# Autodesk Inventor assembly: CARCASA_ESTRUCTURA_Y_CHAPAS
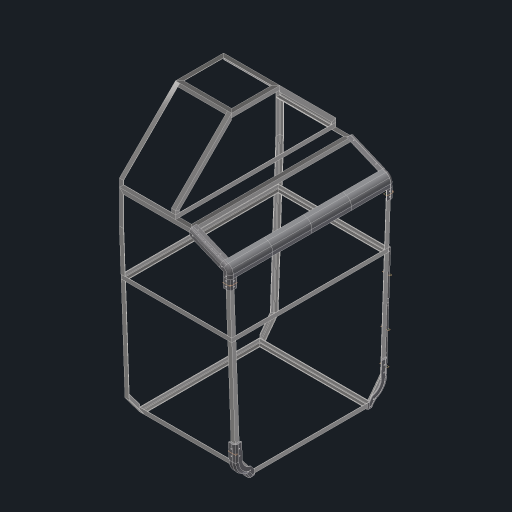
[picture p0: Inventor's stored thumbnail of the model, 512x512]
Saved by Autodesk Inventor 2024.3 (Build 283343000, 343)
## iProperties
Created: 2024-05-18
Part Number: CARCASA_ESTRUCTURA_Y_CHAPAS
Material: Generic
Document SubType Name: Assembly
Designer: Niler
Author: Niler
## Documents named in this file (17)
- C:\Users\Niler\OneDrive\Escritorio\RECICLADOR\RECICLADOR_MODELO_3D\VERSION_3_COMPLETA\CARCASA_ESTRUCTURA_Y_CHAPAS.iam
- C:\Users\Niler\OneDrive\Escritorio\RECICLADOR\RECICLADOR_MODELO_3D\VERSION_3_COMPLETA\ESTRUCTURA\ESTRUCTURA_COMPLETA.iam
- C:\Users\Niler\OneDrive\Escritorio\RECICLADOR\RECICLADOR_MODELO_3D\VERSION_3_COMPLETA\ESQUINAS\ESQUINA_REDONDEADA_R20_P1.ipt
- C:\Users\Niler\OneDrive\Escritorio\RECICLADOR\RECICLADOR_MODELO_3D\VERSION_3_COMPLETA\ESQUINAS\ESQUINA_REDONDEADA_R20_P2.ipt
- C:\Users\Niler\OneDrive\Escritorio\RECICLADOR\RECICLADOR_MODELO_3D\VERSION_3_COMPLETA\ESQUINAS\ESQUINA_REDONDEADA_R20_P3.ipt
- C:\Users\Niler\OneDrive\Escritorio\RECICLADOR\RECICLADOR_MODELO_3D\VERSION_3_COMPLETA\ESQUINAS\ESQUINA_REDONDEADA_R50.ipt
- C:\Users\Niler\OneDrive\Escritorio\RECICLADOR\RECICLADOR_MODELO_3D\VERSION_3_COMPLETA\ESQUINAS\ESQUINA_REDONDEADA_R50_P2.ipt
- C:\Users\Niler\OneDrive\Escritorio\RECICLADOR\RECICLADOR_MODELO_3D\VERSION_3_COMPLETA\ESQUINAS\ESQUINA_REDONDEADA_R20_P4.ipt
- C:\Users\Niler\OneDrive\Escritorio\RECICLADOR\RECICLADOR_MODELO_3D\VERSION_3_COMPLETA\ESQUINAS\ESQUINA_REDONDEADA_R20_P8.ipt
- C:\Users\Niler\OneDrive\Escritorio\RECICLADOR\RECICLADOR_MODELO_3D\VERSION_3_COMPLETA\ESQUINAS\ESQUINA_REDONDEADA_R20_P9.ipt
- C:\Users\Niler\OneDrive\Escritorio\RECICLADOR\RECICLADOR_MODELO_3D\VERSION_3_COMPLETA\ESQUINAS\ESQUINA_REDONDEADA_R20_P5_MIR.ipt
- C:\Users\Niler\OneDrive\Escritorio\RECICLADOR\RECICLADOR_MODELO_3D\VERSION_3_COMPLETA\ESQUINAS\ESQUINA_REDONDEADA_R20_P8_MIR.ipt
- C:\Users\Niler\OneDrive\Escritorio\RECICLADOR\RECICLADOR_MODELO_3D\VERSION_3_COMPLETA\ESQUINAS\ESQUINA_REDONDEADA_R20_P9_MIR.ipt
- C:\Users\Niler\OneDrive\Escritorio\RECICLADOR\RECICLADOR_MODELO_3D\VERSION_3_COMPLETA\ESQUINAS\ESQUINA_REDONDEADA_R20_P1_MIR1.ipt
- C:\Users\Niler\OneDrive\Escritorio\RECICLADOR\RECICLADOR_MODELO_3D\VERSION_3_COMPLETA\ESQUINAS\ESQUINA_REDONDEADA_R20_P2_MIR1.ipt
- C:\Users\Niler\OneDrive\Escritorio\RECICLADOR\RECICLADOR_MODELO_3D\VERSION_3_COMPLETA\ESQUINAS\ESQUINA_REDONDEADA_R20_P3_MIR1.ipt
- C:\Users\Niler\OneDrive\Escritorio\RECICLADOR\RECICLADOR_MODELO_3D\VERSION_3_COMPLETA\ESQUINAS\ESQUINA_REDONDEADA_R20_P4_MIR1.ipt
## Components (25 placed, 16 different names)
1. ESTRUCTURA_COMPLETA:1 [sub-assembly] — Mate:2, Angle:1, Mate:3, Angle:2, Mate:9, Mate:10, Mate:11, Mate:31, Mate:41, Mate:54, Mate:55, Mate:56, Mate:99, Mate:100
2. ESQUINA_REDONDEADA_R20_P1:1 — Mate:2, Angle:1, Mate:4, Mate:30
3. ESQUINA_REDONDEADA_R20_P2:1 — Mate:3, Angle:2, Mate:4, Mate:29
4. ESQUINA_REDONDEADA_R20_P3:1 — Mate:9, Mate:10, Mate:11, Mate:29, Mate:30, Mate:32, Flush:6, Mate:42, Mate:98
5. ESQUINA_REDONDEADA_R20_P4:1 — Mate:31, Mate:32, Flush:6, Mate:40
6. ESQUINA_REDONDEADA_R20_P4:2 — Mate:40, Mate:41, Mate:42
7. ESQUINA_REDONDEADA_R20_P8:1 — Mate:54, Mate:55, Mate:57
8. ESQUINA_REDONDEADA_R20_P9:1 — Mate:56, Mate:57
9. ESQUINA_REDONDEADA_R20_P5_MIR:3 — Mate:66, Flush:11
10. ESQUINA_REDONDEADA_R20_P5_MIR:5 — Mate:66, Flush:11, Flush:13
11. ESQUINA_REDONDEADA_R20_P8_MIR:1 — Flush:13, Mate:70
12. ESQUINA_REDONDEADA_R20_P9_MIR:1 — Mate:70
13. ESQUINA_REDONDEADA_R50_P2:1 — Mate:81, Flush:15, Mate:82, Mate:85, Mate:86, Mate:100
14. ESQUINA_REDONDEADA_R50:1 — Mate:81, Flush:15, Mate:82, Mate:87, Mate:98, Mate:99
15. ESQUINA_REDONDEADA_R50_P2:2 — Mate:85, Mate:86, Mate:95, Mate:96
16. ESQUINA_REDONDEADA_R50:2 — Mate:87, Mate:97
17. ESQUINA_REDONDEADA_R50_P2:3 — Mate:95, Mate:96
18. ESQUINA_REDONDEADA_R50:3 — Mate:97
19. ESQUINA_REDONDEADA_R50_P2:4
20. ESQUINA_REDONDEADA_R50:4
21. ESQUINA_REDONDEADA_R20_P1_MIR1:1 — Mate:101, Mate:102
22. ESQUINA_REDONDEADA_R20_P2_MIR1:1 — Mate:101, Mate:103
23. ESQUINA_REDONDEADA_R20_P3_MIR1:1 — Mate:102, Mate:103, Flush:19, Mate:104, Mate:105
24. ESQUINA_REDONDEADA_R20_P4_MIR1:1 — Flush:19, Mate:104, Mate:106
25. ESQUINA_REDONDEADA_R20_P4_MIR1:2 — Mate:105, Mate:106
## Relationships (55: Mate 45, Flush 8, Angle 2)
- Mate:2: ESTRUCTURA_COMPLETA:1 ↔ ESQUINA_REDONDEADA_R20_P1:1
- Angle:1 (0 deg): ESTRUCTURA_COMPLETA:1 ↔ ESQUINA_REDONDEADA_R20_P1:1
- Mate:3: ESTRUCTURA_COMPLETA:1 ↔ ESQUINA_REDONDEADA_R20_P2:1
- Angle:2 (0 deg): ESTRUCTURA_COMPLETA:1 ↔ ESQUINA_REDONDEADA_R20_P2:1
- Mate:4: ESQUINA_REDONDEADA_R20_P1:1 ↔ ESQUINA_REDONDEADA_R20_P2:1
- Mate:9: ESTRUCTURA_COMPLETA:1 ↔ ESQUINA_REDONDEADA_R20_P3:1
- Mate:10: ESTRUCTURA_COMPLETA:1 ↔ ESQUINA_REDONDEADA_R20_P3:1
- Mate:11: ESTRUCTURA_COMPLETA:1 ↔ ESQUINA_REDONDEADA_R20_P3:1
- Mate:29: ESQUINA_REDONDEADA_R20_P2:1 ↔ ESQUINA_REDONDEADA_R20_P3:1
- Mate:30: ESQUINA_REDONDEADA_R20_P1:1 ↔ ESQUINA_REDONDEADA_R20_P3:1
- Mate:31: ESTRUCTURA_COMPLETA:1 ↔ ESQUINA_REDONDEADA_R20_P4:1
- Mate:32: ESQUINA_REDONDEADA_R20_P3:1 ↔ ESQUINA_REDONDEADA_R20_P4:1
- Flush:6: ESQUINA_REDONDEADA_R20_P3:1 ↔ ESQUINA_REDONDEADA_R20_P4:1
- Mate:40: ESQUINA_REDONDEADA_R20_P4:1 ↔ ESQUINA_REDONDEADA_R20_P4:2
- Mate:41: ESTRUCTURA_COMPLETA:1 ↔ ESQUINA_REDONDEADA_R20_P4:2
- Mate:42: ESQUINA_REDONDEADA_R20_P3:1 ↔ ESQUINA_REDONDEADA_R20_P4:2
- Mate:54: ESTRUCTURA_COMPLETA:1 ↔ ESQUINA_REDONDEADA_R20_P8:1
- Mate:55: ESTRUCTURA_COMPLETA:1 ↔ ESQUINA_REDONDEADA_R20_P8:1
- Mate:56: ESTRUCTURA_COMPLETA:1 ↔ ESQUINA_REDONDEADA_R20_P9:1
- Mate:57: ESQUINA_REDONDEADA_R20_P8:1 ↔ ESQUINA_REDONDEADA_R20_P9:1
- Mate:66: ESQUINA_REDONDEADA_R20_P5_MIR:3 ↔ ESQUINA_REDONDEADA_R20_P5_MIR:5
- Flush:11: ESQUINA_REDONDEADA_R20_P5_MIR:3 ↔ ESQUINA_REDONDEADA_R20_P5_MIR:5
- Flush:13: ESQUINA_REDONDEADA_R20_P5_MIR:5 ↔ ESQUINA_REDONDEADA_R20_P8_MIR:1
- Mate:70: ESQUINA_REDONDEADA_R20_P8_MIR:1 ↔ ESQUINA_REDONDEADA_R20_P9_MIR:1
- Mate:81: ESQUINA_REDONDEADA_R50_P2:1 ↔ ESQUINA_REDONDEADA_R50:1
- Flush:15: ESQUINA_REDONDEADA_R50_P2:1 ↔ ESQUINA_REDONDEADA_R50:1
- Mate:82: ESQUINA_REDONDEADA_R50_P2:1 ↔ ESQUINA_REDONDEADA_R50:1
- [Mate]: ESQUINA_REDONDEADA_R50_P2:2 ↔ ESQUINA_REDONDEADA_R50:2
- [Flush]: ESQUINA_REDONDEADA_R50_P2:2 ↔ ESQUINA_REDONDEADA_R50:2
- [Mate]: ESQUINA_REDONDEADA_R50_P2:2 ↔ ESQUINA_REDONDEADA_R50:2
- Mate:85: ESQUINA_REDONDEADA_R50_P2:1 ↔ ESQUINA_REDONDEADA_R50_P2:2
- Mate:86: ESQUINA_REDONDEADA_R50_P2:1 ↔ ESQUINA_REDONDEADA_R50_P2:2
- Mate:87: ESQUINA_REDONDEADA_R50:1 ↔ ESQUINA_REDONDEADA_R50:2
- [Mate]: ESQUINA_REDONDEADA_R50_P2:3 ↔ ESQUINA_REDONDEADA_R50:3
- [Flush]: ESQUINA_REDONDEADA_R50_P2:3 ↔ ESQUINA_REDONDEADA_R50:3
- [Mate]: ESQUINA_REDONDEADA_R50_P2:3 ↔ ESQUINA_REDONDEADA_R50:3
- [Mate]: ESQUINA_REDONDEADA_R50_P2:4 ↔ ESQUINA_REDONDEADA_R50:4
- [Flush]: ESQUINA_REDONDEADA_R50_P2:4 ↔ ESQUINA_REDONDEADA_R50:4
- [Mate]: ESQUINA_REDONDEADA_R50_P2:4 ↔ ESQUINA_REDONDEADA_R50:4
- [Mate]: ESQUINA_REDONDEADA_R50_P2:3 ↔ ESQUINA_REDONDEADA_R50_P2:4
- [Mate]: ESQUINA_REDONDEADA_R50_P2:3 ↔ ESQUINA_REDONDEADA_R50_P2:4
- [Mate]: ESQUINA_REDONDEADA_R50:3 ↔ ESQUINA_REDONDEADA_R50:4
- Mate:95: ESQUINA_REDONDEADA_R50_P2:2 ↔ ESQUINA_REDONDEADA_R50_P2:3
- Mate:96: ESQUINA_REDONDEADA_R50_P2:2 ↔ ESQUINA_REDONDEADA_R50_P2:3
- Mate:97: ESQUINA_REDONDEADA_R50:2 ↔ ESQUINA_REDONDEADA_R50:3
- Mate:98: ESQUINA_REDONDEADA_R20_P3:1 ↔ ESQUINA_REDONDEADA_R50:1
- Mate:99: ESTRUCTURA_COMPLETA:1 ↔ ESQUINA_REDONDEADA_R50:1
- Mate:100: ESTRUCTURA_COMPLETA:1 ↔ ESQUINA_REDONDEADA_R50_P2:1
- Mate:101: ESQUINA_REDONDEADA_R20_P1_MIR1:1 ↔ ESQUINA_REDONDEADA_R20_P2_MIR1:1
- Mate:102: ESQUINA_REDONDEADA_R20_P1_MIR1:1 ↔ ESQUINA_REDONDEADA_R20_P3_MIR1:1
- Mate:103: ESQUINA_REDONDEADA_R20_P2_MIR1:1 ↔ ESQUINA_REDONDEADA_R20_P3_MIR1:1
- Flush:19: ESQUINA_REDONDEADA_R20_P3_MIR1:1 ↔ ESQUINA_REDONDEADA_R20_P4_MIR1:1
- Mate:104: ESQUINA_REDONDEADA_R20_P3_MIR1:1 ↔ ESQUINA_REDONDEADA_R20_P4_MIR1:1
- Mate:105: ESQUINA_REDONDEADA_R20_P3_MIR1:1 ↔ ESQUINA_REDONDEADA_R20_P4_MIR1:2
- Mate:106: ESQUINA_REDONDEADA_R20_P4_MIR1:1 ↔ ESQUINA_REDONDEADA_R20_P4_MIR1:2
## Named parameters: d158_d155 = 0 mm, d159_d156 = 0 mm, d160_d157 = 0 mm, d164_d155 = 0 mm, d165_d156 = 0 mm, d166_d157 = 0 mm, d167_d158_d155 = 0 mm, d168_d159_d156 = 0 mm, d169_d160_d157 = 0 mm, d170_d161 = 0 mm, d171_d162 = 0 mm, d172_d163 = 0 mm
